# Autodesk Inventor assembly: HSDL-9100
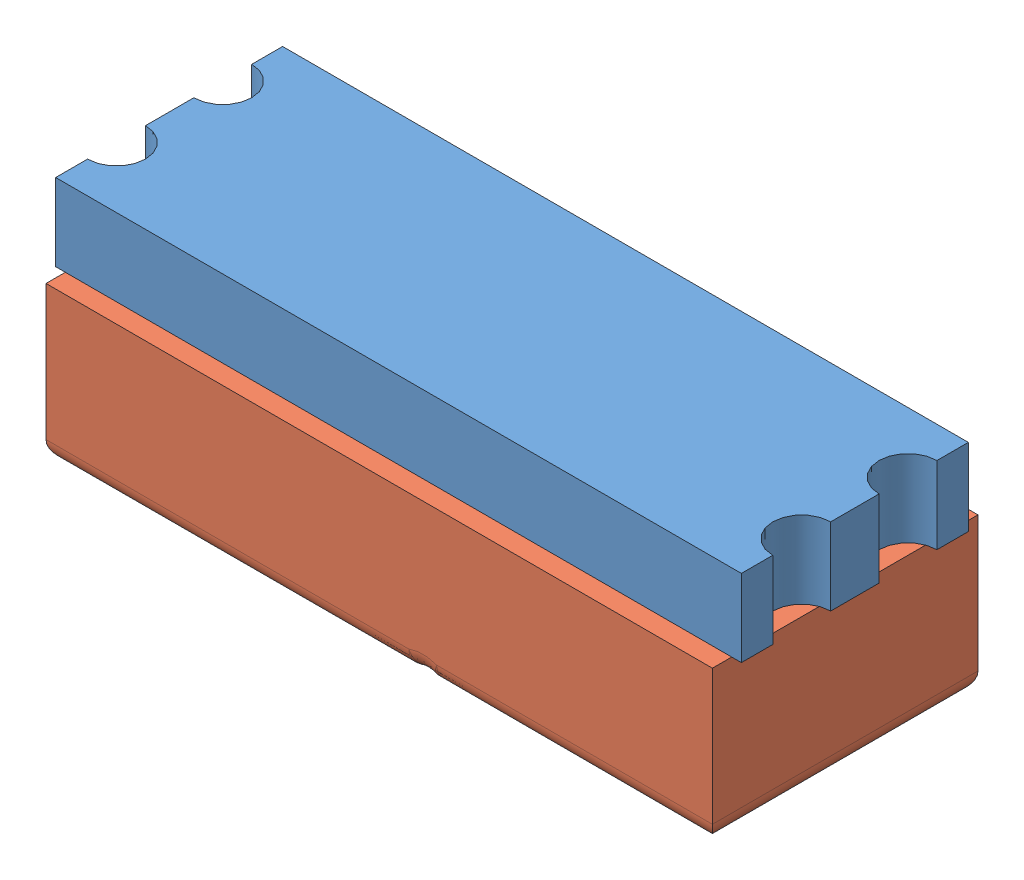
[picture p0: shaded view drawn from the part files that the assembly names]
Saved by Autodesk Inventor 2014 (Build 180170000, 170)
## iProperties
Created: 2013-06-27
Part Number: HSDL-9100
Document SubType Name: Assembly
Designer: hanse
Author: hanse
## Documents named in this file (3)
- C:\Users\Felix\Desktop\Beep\Hardware\3D-CAD\parts\electronic\BEEP\components\HSDL-9100-024\HSDL-9100.iam
- C:\Users\Felix\Desktop\Beep\Hardware\3D-CAD\parts\electronic\BEEP\components\HSDL-9100-024\bottom_pcb.ipt
- C:\Users\Felix\Desktop\Beep\Hardware\3D-CAD\parts\electronic\BEEP\components\HSDL-9100-024\top.ipt
## Components (2 placed, 2 different names)
1. bottom_pcb:1 — Passend:1, Fluchtend:1, Fluchtend:2, Fluchtend:3
2. top:1 — Passend:1, Fluchtend:1, Fluchtend:2, Passend:3, Passend:4
## Relationships (6: Mate 3, Flush 3)
- Passend:1 [Mate]: bottom_pcb:1 ↔ top:1
- Fluchtend:1 [Flush] (-0.2 mm): bottom_pcb:1 ↔ top:1
- Fluchtend:2 [Flush] (0.1 mm): bottom_pcb:1 ↔ top:1
- Passend:3 [Mate] (-3.45 mm): top:1
- Passend:4 [Mate] (-1.375 mm): top:1
- Fluchtend:3 [Flush]: bottom_pcb:1
